# Autodesk Inventor assembly: Odometry module for metal drive train_MIR
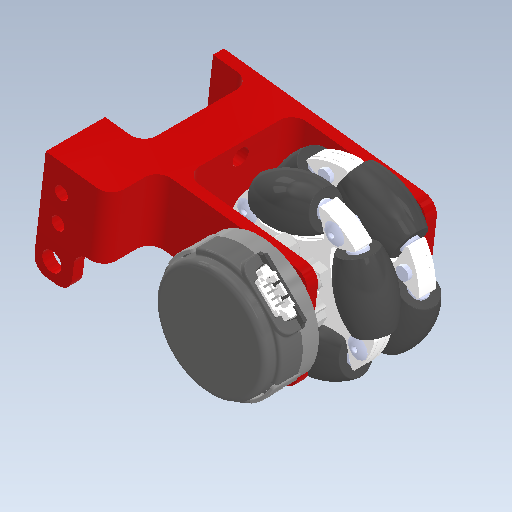
[picture p0: Inventor's stored thumbnail of the model, 512x512]
Saved by Autodesk Inventor 2020 (Build 240168000, 168)
## iProperties
Created: 2019-11-05
Part Number: Odometry module for metal drive train_MIR
Document SubType Name: Assembly
Designer: jackm
Author: ball
## Documents named in this file (8)
- D:\FTC8863\2019 Robot\Odoemetry module\Odometry module for metal drive train_MIR.iam
- D:\FTC8863\2019 Robot\Odoemetry module\Odometry_Holder with motor clearance_MIR.ipt
- D:\FTC8863\Actobotics\535 parts\535042_MIR1.ipt
- D:\FTC8863\Actobotics\634 parts\634064_MIR1.ipt
- D:\FTC8863\2019 Robot\Odoemetry module\wheel_dual_MIR.iam
- D:\FTC8863\2019 Robot\Odoemetry module\E8T-X-250-S-D-D-X_MIR.iam
- D:\FTC8863\2019 Robot\Odoemetry module\90576A161_MEDIUM-STRENGTH STEEL NYLON-INSERT LOCKNUT_MIR1.ipt
- D:\FTC8863\2019 Robot\Odoemetry module\spacer around nuts_MIR.ipt
## Components (9 placed, 7 different names)
1. Odometry_Holder with motor clearance_MIR:1 — Mate:2, Mate:1, Mate:3, Flush:1, Mate:12, Mate:11, Mate:14, Mate:16
2. 535042_MIR1:1 — Mate:2, Mate:1
3. 535042_MIR1:2 — Mate:3, Mate:5
4. 634064_MIR1:1 — Flush:1, Mate:5, Mate:6, Mate:10, Mate:18
5. wheel_dual_MIR:1 [sub-assembly] — Mate:6, Mate:17
6. E8T-X-250-S-D-D-X_MIR:1 [sub-assembly] — Mate:12, Mate:11, Mate:10, Mate:13, Mate:15
7. 90576A161_MEDIUM-STRENGTH STEEL NYLON-INSERT LOCKNUT_MIR1:1 — Mate:14, Mate:13
8. 90576A161_MEDIUM-STRENGTH STEEL NYLON-INSERT LOCKNUT_MIR1:2 — Mate:16, Mate:15
9. spacer around nuts_MIR:1 — Mate:18, Mate:17
## Relationships (15: Mate 14, Flush 1)
- Mate:2: Odometry_Holder with motor clearance_MIR:1 ↔ 535042_MIR1:1
- Mate:1: Odometry_Holder with motor clearance_MIR:1 ↔ 535042_MIR1:1
- Mate:3: Odometry_Holder with motor clearance_MIR:1 ↔ 535042_MIR1:2
- Flush:1: Odometry_Holder with motor clearance_MIR:1 ↔ 634064_MIR1:1
- Mate:5: 535042_MIR1:2 ↔ 634064_MIR1:1
- Mate:6: 634064_MIR1:1 ↔ wheel_dual_MIR:1
- Mate:12: Odometry_Holder with motor clearance_MIR:1 ↔ E8T-X-250-S-D-D-X_MIR:1
- Mate:11: Odometry_Holder with motor clearance_MIR:1 ↔ E8T-X-250-S-D-D-X_MIR:1
- Mate:10: 634064_MIR1:1 ↔ E8T-X-250-S-D-D-X_MIR:1
- Mate:14: Odometry_Holder with motor clearance_MIR:1 ↔ 90576A161_MEDIUM-STRENGTH STEEL NYLON-INSERT LOCKNUT_MIR1:1
- Mate:13: E8T-X-250-S-D-D-X_MIR:1 ↔ 90576A161_MEDIUM-STRENGTH STEEL NYLON-INSERT LOCKNUT_MIR1:1
- Mate:16: Odometry_Holder with motor clearance_MIR:1 ↔ 90576A161_MEDIUM-STRENGTH STEEL NYLON-INSERT LOCKNUT_MIR1:2
- Mate:15: E8T-X-250-S-D-D-X_MIR:1 ↔ 90576A161_MEDIUM-STRENGTH STEEL NYLON-INSERT LOCKNUT_MIR1:2
- Mate:18: 634064_MIR1:1 ↔ spacer around nuts_MIR:1
- Mate:17: wheel_dual_MIR:1 ↔ spacer around nuts_MIR:1
